# Autodesk Inventor assembly: mg996r 3mm frame middle leg
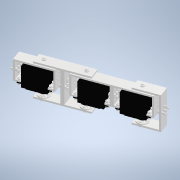
[picture p0: Inventor's stored thumbnail of the model, 180x180]
Saved by Autodesk Inventor 2021.4 (Build 254397000, 397)
## iProperties
Created: 2022-07-09
Part Number: mg996r 3mm frame middle leg
Document SubType Name: Assembly
Designer: isamu
Author: isamu
## Documents named in this file (4)
- D:\personal_projects\robot\inventor\2021\mg996r 3mm frame middle leg.iam
- D:\personal_projects\robot\inventor\2021\base mg996r 3mm frame middle.iam
- D:\personal_projects\robot\exports\screws\m3x8.ipt
- D:\personal_projects\robot\exports\screws\m3 nuts.ipt
## Components (33 placed, 3 different names)
1. base mg996r 3mm frame middle:1 [sub-assembly] — Mate:1, Mate:2, Mate:3, Insert:6, Insert:7, Insert:8, Insert:9, Insert:10, Insert:21, Insert:22, Insert:23, Insert:24, Insert:25
2. base mg996r 3mm frame middle:2 [sub-assembly] — Mate:1, Mate:2, Mate:3, Mate:4, Mate:5, Mate:6, Insert:1, Insert:2, Insert:3, Insert:4, Insert:5, Insert:11, Insert:12, Insert:13, Insert:14, Insert:15
3. base mg996r 3mm frame middle:3 [sub-assembly] — Mate:4, Mate:5, Mate:6, Insert:16, Insert:17, Insert:18, Insert:19, Insert:20, Insert:26, Insert:27, Insert:28, Insert:29, Insert:30
4. m3x8:1 — Insert:5
5. m3x8:2 — Insert:8
6. m3x8:3 — Insert:9
7. m3x8:4 — Insert:3
8. m3x8:5 — Insert:1
9. m3x8:6 — Insert:4
10. m3x8:7 — Insert:2
11. m3x8:8 — Insert:10
12. m3x8:9 — Insert:6
13. m3x8:10 — Insert:7
14. m3 nuts:1 — Insert:15
15. m3 nuts:2 — Insert:16
16. m3 nuts:3 — Insert:13
17. m3 nuts:4 — Insert:17
18. m3 nuts:5 — Insert:18
19. m3 nuts:6 — Insert:14
20. m3 nuts:7 — Insert:12
21. m3 nuts:8 — Insert:11
22. m3 nuts:9 — Insert:19
23. m3 nuts:10 — Insert:20
24. m3x8:11 — Insert:22
25. m3x8:12 — Insert:23
26. m3x8:13 — Insert:25
27. m3x8:14 — Insert:24
28. m3x8:15 — Insert:21
29. m3x8:16 — Insert:28
30. m3x8:17 — Insert:29
31. m3x8:18 — Insert:26
32. m3x8:19 — Insert:27
33. m3x8:20 — Insert:30
## Relationships (36: Insert 30, Mate 6)
- Mate:1: base mg996r 3mm frame middle:1 ↔ base mg996r 3mm frame middle:2
- Mate:2: base mg996r 3mm frame middle:1 ↔ base mg996r 3mm frame middle:2
- Mate:3: base mg996r 3mm frame middle:1 ↔ base mg996r 3mm frame middle:2
- Mate:4: base mg996r 3mm frame middle:2 ↔ base mg996r 3mm frame middle:3
- Mate:5: base mg996r 3mm frame middle:2 ↔ base mg996r 3mm frame middle:3
- Mate:6: base mg996r 3mm frame middle:2 ↔ base mg996r 3mm frame middle:3
- Insert:1: base mg996r 3mm frame middle:2 ↔ m3x8:5
- Insert:2: base mg996r 3mm frame middle:2 ↔ m3x8:7
- Insert:3: base mg996r 3mm frame middle:2 ↔ m3x8:4
- Insert:4: base mg996r 3mm frame middle:2 ↔ m3x8:6
- Insert:5: base mg996r 3mm frame middle:2 ↔ m3x8:1
- Insert:6: base mg996r 3mm frame middle:1 ↔ m3x8:9
- Insert:7: base mg996r 3mm frame middle:1 ↔ m3x8:10
- Insert:8: base mg996r 3mm frame middle:1 ↔ m3x8:2
- Insert:9: base mg996r 3mm frame middle:1 ↔ m3x8:3
- Insert:10: base mg996r 3mm frame middle:1 ↔ m3x8:8
- Insert:11: base mg996r 3mm frame middle:2 ↔ m3 nuts:8
- Insert:12: base mg996r 3mm frame middle:2 ↔ m3 nuts:7
- Insert:13: base mg996r 3mm frame middle:2 ↔ m3 nuts:3
- Insert:14: base mg996r 3mm frame middle:2 ↔ m3 nuts:6
- Insert:15: base mg996r 3mm frame middle:2 ↔ m3 nuts:1
- Insert:16: base mg996r 3mm frame middle:3 ↔ m3 nuts:2
- Insert:17: base mg996r 3mm frame middle:3 ↔ m3 nuts:4
- Insert:18: base mg996r 3mm frame middle:3 ↔ m3 nuts:5
- Insert:19: base mg996r 3mm frame middle:3 ↔ m3 nuts:9
- Insert:20: base mg996r 3mm frame middle:3 ↔ m3 nuts:10
- Insert:21: base mg996r 3mm frame middle:1 ↔ m3x8:15
- Insert:22: base mg996r 3mm frame middle:1 ↔ m3x8:11
- Insert:23: base mg996r 3mm frame middle:1 ↔ m3x8:12
- Insert:24: base mg996r 3mm frame middle:1 ↔ m3x8:14
- Insert:25: base mg996r 3mm frame middle:1 ↔ m3x8:13
- Insert:26: base mg996r 3mm frame middle:3 ↔ m3x8:18
- Insert:27: base mg996r 3mm frame middle:3 ↔ m3x8:19
- Insert:28: base mg996r 3mm frame middle:3 ↔ m3x8:16
- Insert:29: base mg996r 3mm frame middle:3 ↔ m3x8:17
- Insert:30: base mg996r 3mm frame middle:3 ↔ m3x8:20
